# Autodesk Inventor assembly: Joint2
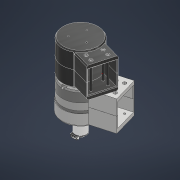
[picture p0: Inventor's stored thumbnail of the model, 180x180]
Saved by Autodesk Inventor 2021 (Build 250183000, 183)
## iProperties
RuleStatus: InUse
Created: 2025-03-14
Part Number: Joint2
Document SubType Name: Assembly
Designer: rocke
Mass: 414.793 g
Surface Area: 1158.92 cm^2
Volume: 253.092 cm^3
Density: 1.6389 g/cm^3
Author: rocke
## Documents named in this file (19)
- C:\Users\rocke\Documents\Robot Arm IPT\Joint2.iam
- C:\Users\rocke\Documents\Robot Arm IPT\Sun Gear.ipt
- C:\Users\rocke\Documents\Robot Arm IPT\Joint2\Design Accelerator\Spur Gears1.iam
- C:\Users\rocke\Documents\Robot Arm IPT\Joint2\Design Accelerator\Spur Gears3.iam
- C:\Users\rocke\Documents\Robot Arm IPT\Planet Carrier.ipt
- C:\Users\rocke\Documents\Robot Arm IPT\Planet Carrier 2.ipt
- C:\Users\rocke\Documents\Robot Arm IPT\Planet Carrier 3.ipt
- C:\Users\rocke\Documents\Inventor\Content Center Files\R2021\en-US\DIN 472(2)\DIN 472 - 16x1.ipt
- C:\Users\rocke\Documents\Inventor\Content Center Files\R2021\en-US\DIN 625 SKF(4)\DIN 625 SKF - SKF 628_8-2Z.ipt
- C:\Users\rocke\Documents\Robot Arm IPT\Ring Cover.ipt
- C:\Users\rocke\Downloads\12V 350RPM Small DFRobot Motor v8.iam
- C:\Users\rocke\Documents\Inventor\Content Center Files\R2021\en-US\ISO 4762(2)\ISO 4762 - M3 x 5ISO.ipt
- C:\Users\rocke\Documents\Robot Arm IPT\Joint2\Design Accelerator\Spur Gear11.ipt
- C:\Users\rocke\Documents\Inventor\Content Center Files\R2021\en-US\GB_T 276-94 60000-2Z\Bearing 61809-2Z GB_T 276-94.ipt
- C:\Users\rocke\Documents\Robot Arm IPT\Ring Cover Top.ipt
- C:\Users\rocke\Documents\Robot Arm IPT\Joint2\Planet Subassembly.iam
- C:\Users\rocke\Downloads\TO-92 flat Formed Leads Horizontal Back.ipt
- C:\Users\rocke\Documents\Robot Arm IPT\Fixation.iam
- C:\Users\rocke\Documents\Robot Arm IPT\Fixation_CPY.iam
## Components (23 placed, 17 different names)
1. Sun Gear:1
2. Spur Gears:1 [sub-assembly]
3. Spur Gears:2 [sub-assembly] — Rotational:4, Rotational:5, Rigid:5
4. Planet Carrier:1 — Rigid:1, Mate:1, Mate:12, Rotational:10, Rotational:11, Rotational:12, Rigid:8
5. Planet Carrier 2:1 — Rigid:1, Mate:2, Mate:11, Rigid:7
6. Planet Carrier 3:1 — Rigid:7, Rotational:13, Rotational:14, Cylindrical:1
7. DIN 625 SKF- with two Z shields SKF 628/8-2Z:1 — Mate:1, Mate:2, Rigid:6, Rotational:9
8. DIN 472 16x1:1 — Rigid:6, Rigid:8
9. Ring Cover:1 — Rotational:2, Rotational:3, Mate:5, Mate:6, Mate:7, Mate:8, Mate:9, Mate:10, Rotational:4, Rotational:5, Insert:1
10. 12V 350RPM Small DFRobot Motor v8:1 [sub-assembly] — Rotational:2, Rotational:3, Rotational:7
11. ISO 4762 M3 x 5:1 — Mate:5, Mate:6
12. ISO 4762 M3 x 5:2 — Mate:7, Mate:8
13. ISO 4762 M3 x 5:3 — Mate:9, Mate:10
14. Spur Gear1:1 — Rotational:7, Rotational:9, Rotation:1, Rotation:2, Rotation:3
15. Rolling bearing GB/T 276-1994 Type 60000-2Z 61809-2Z:1 — Mate:11, Mate:12
16. Rolling bearing GB/T 276-1994 Type 60000-2Z 61809-2Z:2 — Rotational:13
17. Ring Cover Top:1 — Rigid:5, Rigid:9
18. Planet Subassembly:1 [sub-assembly] — Rotational:10, Rotation:1
19. Planet Subassembly:2 [sub-assembly] — Rotational:11, Rotation:3
20. Planet Subassembly:3 [sub-assembly] — Rotational:12, Rotation:2
21. TO-92 flat Formed Leads Horizontal Back:1 — Rigid:9
22. Fixation:1 [sub-assembly] — Rotational:14, Cylindrical:1
23. Fixation_CPY:1 [sub-assembly] — Insert:1
## Relationships (32: RevoluteJoint 11, Mate 10, WeldJoint 6, RelateRotation 3, CylindricalJoint 1, Insert 1)
- Rigid:1 [WeldJoint]: Planet Carrier:1 ↔ Planet Carrier 2:1
- Mate:1: Planet Carrier:1 ↔ DIN 625 SKF- with two Z shields SKF 628/8-2Z:1
- Mate:2: Planet Carrier 2:1 ↔ DIN 625 SKF- with two Z shields SKF 628/8-2Z:1
- Rotational:2 [RevoluteJoint]: Ring Cover:1 ↔ 12V 350RPM Small DFRobot Motor v8:1
- Rotational:3 [RevoluteJoint]: Ring Cover:1 ↔ 12V 350RPM Small DFRobot Motor v8:1
- Mate:5: Ring Cover:1 ↔ ISO 4762 M3 x 5:1
- Mate:6: Ring Cover:1 ↔ ISO 4762 M3 x 5:1
- Mate:7: Ring Cover:1 ↔ ISO 4762 M3 x 5:2
- Mate:8: Ring Cover:1 ↔ ISO 4762 M3 x 5:2
- Mate:9: Ring Cover:1 ↔ ISO 4762 M3 x 5:3
- Mate:10: Ring Cover:1 ↔ ISO 4762 M3 x 5:3
- Rotational:4 [RevoluteJoint]: Spur Gears:2 ↔ Ring Cover:1
- Rotational:5 [RevoluteJoint]: Spur Gears:2 ↔ Ring Cover:1
- Rotational:7 [RevoluteJoint]: 12V 350RPM Small DFRobot Motor v8:1 ↔ Spur Gear1:1
- Mate:11: Planet Carrier 2:1 ↔ Rolling bearing GB/T 276-1994 Type 60000-2Z 61809-2Z:1
- Mate:12: Planet Carrier:1 ↔ Rolling bearing GB/T 276-1994 Type 60000-2Z 61809-2Z:1
- Rigid:5 [WeldJoint]: Spur Gears:2 ↔ Ring Cover Top:1
- Rigid:6 [WeldJoint]: DIN 625 SKF- with two Z shields SKF 628/8-2Z:1 ↔ DIN 472 16x1:1
- Rotational:9 [RevoluteJoint]: DIN 625 SKF- with two Z shields SKF 628/8-2Z:1 ↔ Spur Gear1:1
- Rotational:10 [RevoluteJoint]: Planet Carrier:1 ↔ Planet Subassembly:1
- Rotation:1 [RelateRotation] (1 ul): Spur Gear1:1 ↔ Planet Subassembly:1
- Rotational:11 [RevoluteJoint]: Planet Carrier:1 ↔ Planet Subassembly:2
- Rotational:12 [RevoluteJoint]: Planet Carrier:1 ↔ Planet Subassembly:3
- Rotation:2 [RelateRotation] (1 ul): Spur Gear1:1 ↔ Planet Subassembly:3
- Rotation:3 [RelateRotation] (1 ul): Spur Gear1:1 ↔ Planet Subassembly:2
- Rigid:7 [WeldJoint]: Planet Carrier 2:1 ↔ Planet Carrier 3:1
- Rotational:13 [RevoluteJoint]: Planet Carrier 3:1 ↔ Rolling bearing GB/T 276-1994 Type 60000-2Z 61809-2Z:2
- Rigid:8 [WeldJoint]: Planet Carrier:1 ↔ DIN 472 16x1:1
- Rigid:9 [WeldJoint]: Ring Cover Top:1 ↔ TO-92 flat Formed Leads Horizontal Back:1
- Rotational:14 [RevoluteJoint]: Planet Carrier 3:1 ↔ Fixation:1
- Cylindrical:1: Planet Carrier 3:1 ↔ Fixation:1
- Insert:1: Ring Cover:1 ↔ Fixation_CPY:1
